# Autodesk Inventor assembly: zloz_2
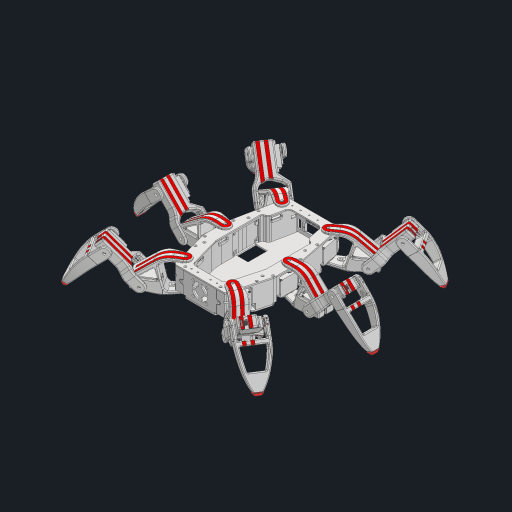
[picture p0: Inventor's stored thumbnail of the model, 512x512]
Saved by Autodesk Inventor 2023.4 (Build 274418000, 418)
## iProperties
Created: 2024-07-26
Part Number: zloz_2
Document SubType Name: Assembly
Designer: kamil
Author: kamil
## Documents named in this file (17)
- E:\PROJECTS_REPOS\Robal-2.0\mechanics\zloz_2.iam
- E:\PROJECTS_REPOS\Robal-2.0\mechanics\Sub-Assy Buck Converter.ipt
- E:\PROJECTS_REPOS\Robal-2.0\mechanics\li_pol_3S_5000mAh.ipt
- E:\PROJECTS_REPOS\Robal-2.0\mechanics\uchwyt_serwa_podwojny.ipt
- E:\PROJECTS_REPOS\Robal-2.0\mechanics\uchwyt_serwa_podwojny_MIR.ipt
- E:\PROJECTS_REPOS\Robal-2.0\mechanics\dol.ipt
- E:\PROJECTS_REPOS\Robal-2.0\mechanics\gora.ipt
- E:\PROJECTS_REPOS\Robal-2.0\mechanics\pokrywa_tyl.ipt
- E:\PROJECTS_REPOS\Robal-2.0\mechanics\pokrywa_przod.ipt
- E:\PROJECTS_REPOS\Robal-2.0\mechanics\noga_pre.iam
- E:\PROJECTS_REPOS\Robal-2.0\mechanics\Standard-Servo.ipt
- E:\PROJECTS_REPOS\Robal-2.0\mechanics\uchwyt_li_pol.ipt
- E:\PROJECTS_REPOS\Robal-2.0\mechanics\pokrywa_gora.ipt
- E:\PROJECTS_REPOS\Robal-2.0\mechanics\RPI_2.iam
- E:\PROJECTS_REPOS\Robal-2.0\mechanics\Standard-Servo_MIR1.ipt
- E:\PROJECTS_REPOS\Robal-2.0\mechanics\step\robal_power_board_new\robal_power_board_new.ipt
- E:\PROJECTS_REPOS\Robal-2.0\mechanics\noga_pre_MIR2.iam
## Components (25 placed, 16 different names)
1. Sub-Assy Buck Converter:1 — Mate:20, Mate:24, Mate:25
2. li_pol_3S_5000mAh:1 — Zestawiające:48, Zestawiające:49, Mate:77, Flush:17
3. uchwyt_serwa_podwojny:1 — Mate:14, Mate:15, Mate:16, Mate:20, Mate:21, Mate:24, Mate:25, Flush:13, Mate:33, Równoległe:14, Symetria:1, Flush:15, Mate:60, Mate:63
4. uchwyt_serwa_podwojny_MIR:1 — Mate:17, Mate:22, Mate:23, Mate:26, Mate:27, Mate:28, Mate:34, Mate:38, Angle:1, Mate:44, Mate:45, Symetria:1, Mate:61, Mate:64, Mate:66, Mate:67, Mate:68, Mate:69, Mate:70
5. dol:1 — Mate:11, Mate:12, Mate:13, Mate:14, Mate:15, Mate:16, Mate:17, Zestawiające:48
6. gora:1 — Mate:21, Mate:22, Mate:23, Mate:39, Mate:40, Mate:41, Mate:42, Mate:43, Równoległe:14, Zestawiające:53, Zestawiające:54, Mate:62
7. Sub-Assy Buck Converter:2 — Mate:26, Mate:27, Mate:28
8. pokrywa_tyl:1 — Flush:15, Mate:60, Mate:61, Mate:81
9. pokrywa_przod:1 — Flush:13, Mate:33, Mate:34
10. noga_pre:1 [sub-assembly] — Mate:38, Mate:39, Mate:46
11. noga_pre:2 [sub-assembly] — Mate:40, Mate:41, Mate:65
12. noga_pre:3 [sub-assembly] — Mate:42, Mate:43
13. Standard-Servo:1 — Angle:1, Mate:44, Mate:45, Mate:46
14. uchwyt_li_pol:1 — Zestawiające:49, Flush:16, Mate:77, Mate:78, Mate:79, Mate:80, Mate:81, Flush:17
15. pokrywa_gora:1 — Zestawiające:53, Zestawiające:54
16. RPI_2:1 [sub-assembly] — Mate:62, Mate:63, Mate:64
17. Standard-Servo:2 — Mate:65, Mate:66, Mate:67
18. Standard-Servo:3 — Mate:68, Mate:69, Mate:70
19. Standard-Servo_MIR1:1
20. Standard-Servo_MIR1:2
21. Standard-Servo_MIR1:3
22. robal_power_board_new:1 — Mate:78, Mate:79, Mate:80
23. noga_pre_MIR2:1 [sub-assembly]
24. noga_pre_MIR2:2 [sub-assembly]
25. noga_pre_MIR2:3 [sub-assembly]
## Relationships (54: Mate 47, Flush 5, Angle 1, Symmetry 1)
- Mate:11 (-31.7995 mm): dol:1
- Mate:12: dol:1
- Mate:13: dol:1
- Mate:14: uchwyt_serwa_podwojny:1 ↔ dol:1
- Mate:15: uchwyt_serwa_podwojny:1 ↔ dol:1
- Mate:16: uchwyt_serwa_podwojny:1 ↔ dol:1
- Mate:17: uchwyt_serwa_podwojny_MIR:1 ↔ dol:1
- Mate:20: Sub-Assy Buck Converter:1 ↔ uchwyt_serwa_podwojny:1
- Mate:21: uchwyt_serwa_podwojny:1 ↔ gora:1
- Mate:22: uchwyt_serwa_podwojny_MIR:1 ↔ gora:1
- Mate:23: uchwyt_serwa_podwojny_MIR:1 ↔ gora:1
- Mate:24: Sub-Assy Buck Converter:1 ↔ uchwyt_serwa_podwojny:1
- Mate:25: Sub-Assy Buck Converter:1 ↔ uchwyt_serwa_podwojny:1
- Mate:26: uchwyt_serwa_podwojny_MIR:1 ↔ Sub-Assy Buck Converter:2
- Mate:27: uchwyt_serwa_podwojny_MIR:1 ↔ Sub-Assy Buck Converter:2
- Mate:28: uchwyt_serwa_podwojny_MIR:1 ↔ Sub-Assy Buck Converter:2
- Flush:13: uchwyt_serwa_podwojny:1 ↔ pokrywa_przod:1
- Mate:33: uchwyt_serwa_podwojny:1 ↔ pokrywa_przod:1
- Mate:34: uchwyt_serwa_podwojny_MIR:1 ↔ pokrywa_przod:1
- Mate:38: uchwyt_serwa_podwojny_MIR:1 ↔ noga_pre:1
- Mate:39: gora:1 ↔ noga_pre:1
- Mate:40: gora:1 ↔ noga_pre:2
- Mate:41: gora:1 ↔ noga_pre:2
- Mate:42: gora:1 ↔ noga_pre:3
- Mate:43: gora:1 ↔ noga_pre:3
- Angle:1 (180 deg): uchwyt_serwa_podwojny_MIR:1 ↔ Standard-Servo:1
- Mate:44: uchwyt_serwa_podwojny_MIR:1 ↔ Standard-Servo:1
- Mate:45: uchwyt_serwa_podwojny_MIR:1 ↔ Standard-Servo:1
- Mate:46: noga_pre:1 ↔ Standard-Servo:1
- Równoległe:14 [Flush]: uchwyt_serwa_podwojny:1 ↔ gora:1
- Symetria:1 [Symmetry]: uchwyt_serwa_podwojny:1 ↔ uchwyt_serwa_podwojny_MIR:1
- Zestawiające:48 [Mate]: li_pol_3S_5000mAh:1 ↔ dol:1
- Zestawiające:49 [Mate]: li_pol_3S_5000mAh:1 ↔ uchwyt_li_pol:1
- Zestawiające:53 [Mate]: gora:1 ↔ pokrywa_gora:1
- Zestawiające:54 [Mate]: gora:1 ↔ pokrywa_gora:1
- Flush:15: uchwyt_serwa_podwojny:1 ↔ pokrywa_tyl:1
- Mate:60: uchwyt_serwa_podwojny:1 ↔ pokrywa_tyl:1
- Mate:61: uchwyt_serwa_podwojny_MIR:1 ↔ pokrywa_tyl:1
- Mate:62: gora:1 ↔ RPI_2:1
- Mate:63: uchwyt_serwa_podwojny:1 ↔ RPI_2:1
- Mate:64: uchwyt_serwa_podwojny_MIR:1 ↔ RPI_2:1
- Mate:65: noga_pre:2 ↔ Standard-Servo:2
- Mate:66 (0.8 mm): uchwyt_serwa_podwojny_MIR:1 ↔ Standard-Servo:2
- Mate:67: uchwyt_serwa_podwojny_MIR:1 ↔ Standard-Servo:2
- Mate:68: uchwyt_serwa_podwojny_MIR:1 ↔ Standard-Servo:3
- Mate:69: uchwyt_serwa_podwojny_MIR:1 ↔ Standard-Servo:3
- Mate:70 (0.8 mm): uchwyt_serwa_podwojny_MIR:1 ↔ Standard-Servo:3
- Flush:16 (25.5 mm): uchwyt_li_pol:1
- Mate:77: li_pol_3S_5000mAh:1 ↔ uchwyt_li_pol:1
- Mate:78: uchwyt_li_pol:1 ↔ robal_power_board_new:1
- Mate:79: uchwyt_li_pol:1 ↔ robal_power_board_new:1
- Mate:80: uchwyt_li_pol:1 ↔ robal_power_board_new:1
- Mate:81 (15 mm): pokrywa_tyl:1 ↔ uchwyt_li_pol:1
- Flush:17: li_pol_3S_5000mAh:1 ↔ uchwyt_li_pol:1
